# Autodesk Inventor assembly: lower_bulkhead
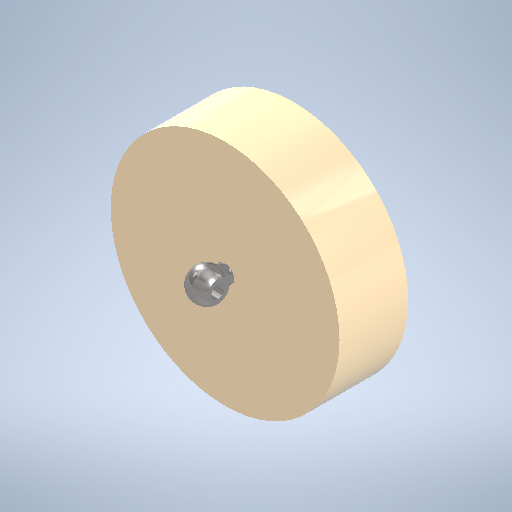
[picture p0: Inventor's stored thumbnail of the model, 512x512]
Saved by Autodesk Inventor 2025 (Build 290162010, 162A)
## iProperties
Created: 2024-07-19
Part Number: lower_bulkhead
Document SubType Name: Assembly
Designer: HP
Author: HP
## Documents named in this file (5)
- C:\Users\HP\Desktop\Project CAD files\lower_bulkhead.iam
- C:\Users\HP\Desktop\Project CAD files\lower_bulkhead.ipt
- C:\Users\HP\Documents\Inventor\Content Center Files\R2025\en-US\GB 798-88\Eye bolt GB 798 M8 x 50.ipt
- C:\Users\HP\Documents\Inventor\Content Center Files\R2025\en-US\AS 1237 (3.1)\AS 1237 - 8 mm(1)Aluminium-6061.ipt
- C:\Users\HP\Documents\Inventor\Content Center Files\R2025\en-US\BS EN 24032\ISO 4032 - M8BS EN.ipt
## Components (4 placed, 4 different names)
1. lower_bulkhead:1 — Insert:1, Mate:2
2. Bolt GB/T 798-1988 M8 x 50:1 — Insert:1, Mate:1, Mate:3
3. AS 1237 (3.1) 8 mm - Aluminum 6061:1 — Mate:1, Mate:2, Mate:4
4. BS EN 24032 - Metric M8:1 — Mate:3, Mate:4
## Relationships (5: Mate 4, Insert 1)
- Insert:1 (-20 mm): lower_bulkhead:1 ↔ Bolt GB/T 798-1988 M8 x 50:1
- Mate:1: Bolt GB/T 798-1988 M8 x 50:1 ↔ AS 1237 (3.1) 8 mm - Aluminum 6061:1
- Mate:2: lower_bulkhead:1 ↔ AS 1237 (3.1) 8 mm - Aluminum 6061:1
- Mate:3: Bolt GB/T 798-1988 M8 x 50:1 ↔ BS EN 24032 - Metric M8:1
- Mate:4: AS 1237 (3.1) 8 mm - Aluminum 6061:1 ↔ BS EN 24032 - Metric M8:1
